# Autodesk Inventor assembly: 1603A270_UNFINISHED BRASS SURFACE-MNT HINGE WHOLES ASSEMBLY
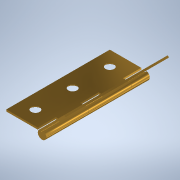
[picture p0: Inventor's stored thumbnail of the model, 180x180]
Saved by Autodesk Inventor 2021 (Build 250183000, 183)
## iProperties
Created: 2021-05-17
Part Number: 1603A270_UNFINISHED BRASS SURFACE-MNT HINGE WHOLES ASSEMBLY
Document SubType Name: Assembly
Designer: Barksdale
Author: Barksdale
## Documents named in this file (3)
- C:\Users\Barksdale\Dropbox (MIT)\MPI Group Folder\MPS\MPSV2\McMaster Carr Parts\1603A270_UNFINISHED BRASS SURFACE-MNT HINGE WHOLES ASSEMBLY.iam
- C:\Users\Barksdale\Dropbox (MIT)\MPI Group Folder\MPS\MPSV2\McMaster Carr Parts\1603A270_UNFINISHED BRASS SURFACE-MNT HINGE WHOLES_A.ipt
- C:\Users\Barksdale\Dropbox (MIT)\MPI Group Folder\MPS\MPSV2\McMaster Carr Parts\1603A270_UNFINISHED BRASS SURFACE-MNT HINGE WHOLES_B.ipt
## Components (2 placed, 2 different names)
1. 1603A270_UNFINISHED BRASS SURFACE-MNT HINGE WHOLES_A:1 — Mate:1, Mate:2, Angle:1
2. 1603A270_UNFINISHED BRASS SURFACE-MNT HINGE WHOLES_B:1 — Mate:1, Mate:2, Angle:1
## Relationships (3: Mate 2, Angle 1)
- Mate:1: 1603A270_UNFINISHED BRASS SURFACE-MNT HINGE WHOLES_A:1 ↔ 1603A270_UNFINISHED BRASS SURFACE-MNT HINGE WHOLES_B:1
- Mate:2: 1603A270_UNFINISHED BRASS SURFACE-MNT HINGE WHOLES_A:1 ↔ 1603A270_UNFINISHED BRASS SURFACE-MNT HINGE WHOLES_B:1
- Angle:1 (45 deg): 1603A270_UNFINISHED BRASS SURFACE-MNT HINGE WHOLES_A:1 ↔ 1603A270_UNFINISHED BRASS SURFACE-MNT HINGE WHOLES_B:1
